# Autodesk Inventor assembly: Złożenie całości
(part 2 of 2)
- Wstaw:98 [Insert]: Prowadnica liniowa typu MGN12H 600mm:1 ↔ CNS 3932 M 3 x 5:80
- Wstaw:99 [Insert]: Prowadnica liniowa typu MGN12H 600mm:1 ↔ CNS 3932 M 3 x 5:81
- Wstaw:100 [Insert]: Prowadnica liniowa typu MGN12H 600mm:1 ↔ CNS 3932 M 3 x 5:82
- Wstaw:101 [Insert]: Prowadnica liniowa typu MGN12H 600mm:1 ↔ CNS 3932 M 3 x 5:83
- Wstaw:102 [Insert]: Prowadnica liniowa typu MGN12H 600mm:1 ↔ CNS 3932 M 3 x 5:84
- Zestawiający:70 [Mate]: Prowadnica liniowa typu MGN12H 600mm:2 ↔ Wózek MGN12H:1
- Zestawiający:71 [Mate]: Prowadnica liniowa typu MGN12H 600mm:2 ↔ Wózek MGN12H:1
- Zestawiający:72 [Mate]: Prowadnica liniowa typu MGN12H 600mm:1 ↔ Wózek MGN12H:2
- Zestawiający:73 [Mate]: Prowadnica liniowa typu MGN12H 600mm:1 ↔ Wózek MGN12H:2
- Równoległy:56 [Flush]: Wózek MGN12H:1 ↔ Wózek MGN12H:2
- Zestawiający:77 [Mate]: Profil dolny posuwu osi Y:1 ↔ Wspornik pionowy osi Y - lewa strona:1
- Równoległy:57 [Flush]: Profil dolny posuwu osi Y:1 ↔ Wspornik pionowy osi Y - lewa strona:1
- Równoległy:58 [Flush]: Profil dolny posuwu osi Y:1 ↔ Wspornik pionowy osi Y - lewa strona:1
- Zestawiający:78 [Mate]: Łożysko kulowe jednorzędowe 6200 2RS:1 ↔ Wspornik pionowy osi Y - lewa strona:1
- Równoległy:59 [Flush]: Łożysko kulowe jednorzędowe 6200 2RS:1 ↔ Wspornik pionowy osi Y - lewa strona:1
- Zestawiający:79 [Mate]: Profil dolny posuwu osi Y:1 ↔ Wspornik pionowy osi Y - prawa strona:1
- Równoległy:60 [Flush]: Profil dolny posuwu osi Y:1 ↔ Wspornik pionowy osi Y - prawa strona:1
- Równoległy:61 [Flush]: Profil dolny posuwu osi Y:1 ↔ Wspornik pionowy osi Y - prawa strona:1
- Równoległy:63 [Flush]: Profil aluminiowy alutec K&K 104080:1 ↔ Prowadnica liniowa typu MGN12H 600mm:2
- Równoległy:64 [Flush]: Profil aluminiowy alutec K&K 104080:1 ↔ Prowadnica liniowa typu MGN12H 600mm:1
- Zestawiający:80 [Mate]: Wózek MGN9C:1 ↔ Wspornik pionowy osi Y - lewa strona:1
- Zestawiający:81 [Mate]: Wózek MGN9C:2 ↔ Wspornik pionowy osi Y - lewa strona:1
- Zestawiający:82 [Mate]: Wózek MGN9C:3 ↔ Wspornik pionowy osi Y - prawa strona:1
- Zestawiający:83 [Mate]: Wózek MGN9C:4 ↔ Wspornik pionowy osi Y - prawa strona:1
- Zestawiający:84 [Mate]: Profil aluminiowy alutec K&K 104080:1 ↔ Wspornik pionowy osi Y - prawa strona:1
- Równoległy:65 [Flush] (70 mm): Profil aluminiowy alutec K&K 104080:1 ↔ Wspornik pionowy osi Y - prawa strona:1
- Równoległy:66 [Flush]: Profil aluminiowy alutec K&K 104080:1 ↔ Wspornik pionowy osi Y - prawa strona:1
- Zestawiający:94 [Mate] (70 mm): Wrzeciono Elektrowrzeciono CNC 0.8kw:1 ↔ Sklejka stołu:1
- Równoległy:67 [Flush]: Wspornik pionowy osi Y - prawa strona:1 ↔ Wspornik łożyska osi Y - prawa strona:1
- Zestawiający:97 [Mate]: Wspornik pionowy osi Y - prawa strona:1 ↔ Wspornik łożyska osi Y - prawa strona:1
- Równoległy:68 [Flush]: Wspornik pionowy osi Y - prawa strona:1 ↔ Wspornik łożyska osi Y - prawa strona:1
- Zestawiający:106 [Mate]: Wspornik pionowy osi Z:1 ↔ Obudowa nakrętki trapezowej fi 16:2
- Zestawiający:107 [Mate]: Wspornik pionowy osi Z:1 ↔ Obudowa nakrętki trapezowej fi 16:2
- Zestawiający:108 [Mate]: Wspornik pionowy osi Z:1 ↔ Obudowa nakrętki trapezowej fi 16:2
- Zestawiający:109 [Mate]: Nakrętka trapezowa kołnierzowa JFRM-2835TR16x4:2 ↔ Obudowa nakrętki trapezowej fi 16:2
- Zestawiający:110 [Mate]: Nakrętka trapezowa kołnierzowa JFRM-2835TR16x4:2 ↔ Obudowa nakrętki trapezowej fi 16:2
- Zestawiający:111 [Mate]: Nakrętka trapezowa kołnierzowa JFRM-2835TR16x4:2 ↔ Obudowa nakrętki trapezowej fi 16:2
- Zestawiający:112 [Mate]: Nakrętka trapezowa kołnierzowa JFRM-2835TR16x4:1 ↔ Obudowa nakrętki trapezowej fi 16:1
- Wstaw:111 [Insert]: Nakrętka trapezowa kołnierzowa JFRM-2835TR16x4:2 ↔ CNS 3932 M 5 x 10:9
- Wstaw:112 [Insert]: Nakrętka trapezowa kołnierzowa JFRM-2835TR16x4:2 ↔ CNS 3932 M 5 x 10:10
- Wstaw:113 [Insert]: Nakrętka trapezowa kołnierzowa JFRM-2835TR16x4:2 ↔ CNS 3932 M 5 x 10:11
- Wstaw:114 [Insert]: Nakrętka trapezowa kołnierzowa JFRM-2835TR16x4:2 ↔ CNS 3932 M 5 x 10:12
- Wstaw:115 [Insert]: Nakrętka trapezowa kołnierzowa JFRM-2835TR16x4:2 ↔ CNS 3932 M 5 x 10:13
- Wstaw:116 [Insert]: Nakrętka trapezowa kołnierzowa JFRM-2835TR16x4:2 ↔ CNS 3932 M 5 x 10:14
- Wstaw:117 [Insert]: Nakrętka trapezowa kołnierzowa JFRM-2835TR16x4:1 ↔ CNS 3932 M 5 x 10:15
- Wstaw:118 [Insert]: Nakrętka trapezowa kołnierzowa JFRM-2835TR16x4:1 ↔ CNS 3932 M 5 x 10:16
- Wstaw:119 [Insert]: Nakrętka trapezowa kołnierzowa JFRM-2835TR16x4:1 ↔ CNS 3932 M 5 x 10:17
- Wstaw:120 [Insert]: Nakrętka trapezowa kołnierzowa JFRM-2835TR16x4:1 ↔ CNS 3932 M 5 x 10:18
- Wstaw:121 [Insert]: Nakrętka trapezowa kołnierzowa JFRM-2835TR16x4:1 ↔ CNS 3932 M 5 x 10:19
- Wstaw:122 [Insert]: Nakrętka trapezowa kołnierzowa JFRM-2835TR16x4:1 ↔ CNS 3932 M 5 x 10:20
- Wstaw:123 [Insert]: Obudowa nakrętki trapezowej fi 16:2 ↔ CNS 3932 M 5 x 12:5
- Wstaw:124 [Insert]: Obudowa nakrętki trapezowej fi 16:2 ↔ CNS 3932 M 5 x 12:8
- Wstaw:125 [Insert]: Obudowa nakrętki trapezowej fi 16:2 ↔ CNS 3932 M 5 x 12:6
- Wstaw:126 [Insert]: Obudowa nakrętki trapezowej fi 16:2 ↔ CNS 3932 M 5 x 12:7
- Wstaw:127 [Insert]: Tuleja zaciskowo rozprężna RCK BK 80 8x15 Clampex:2 ↔ CNS 3932 M 4 x 6:7
- Wstaw:128 [Insert]: Tuleja zaciskowo rozprężna RCK BK 80 8x15 Clampex:2 ↔ CNS 3932 M 4 x 6:8
- Wstaw:129 [Insert]: Tuleja zaciskowo rozprężna RCK BK 80 8x15 Clampex:2 ↔ CNS 3932 M 4 x 6:9
- Wstaw:130 [Insert]: Tuleja zaciskowo rozprężna RCK BK 80 8x15 Clampex:2 ↔ CNS 3932 M 4 x 6:10
- Wstaw:131 [Insert]: Tuleja zaciskowo rozprężna RCK BK 80 8x15 Clampex:2 ↔ CNS 3932 M 4 x 6:11
- Wstaw:132 [Insert]: Tuleja zaciskowo rozprężna RCK BK 80 8x15 Clampex:2 ↔ CNS 3932 M 4 x 6:12
- Zestawiający:118 [Mate]: Silnik krokowy SM 60 100-4004AF - 4Nm:2 ↔ Koło zębate 21 T5 14 2F:2
- Zestawiający:119 [Mate] (1 mm): Silnik krokowy SM 60 100-4004AF - 4Nm:2 ↔ Koło zębate 21 T5 14 2F:2
- Zestawiający:120 [Mate] (18 mm): Wspornik pionowy osi Y - prawa strona:1 ↔ Silnik krokowy SM 60 100-4004AF - 4Nm:2
- Wstaw:133 [Insert]: Wspornik pionowy osi Y - lewa strona:1 ↔ CNS 3932 M 8 x 14:1
- Wstaw:134 [Insert]: Wspornik pionowy osi Y - lewa strona:1 ↔ CNS 3932 M 8 x 14:2
- Wstaw:135 [Insert]: Wspornik pionowy osi Y - prawa strona:1 ↔ CNS 3932 M 8 x 14:3
- Wstaw:136 [Insert]: Wspornik pionowy osi Y - prawa strona:1 ↔ CNS 3932 M 8 x 14:4
- Zestawiający:135 [Mate]: Profil dolny długi:2 ↔ Profil dolny krótki:2
- Wstaw:145 [Insert]: Wspornik pionowy osi Y - prawa strona:1 ↔ CNS 3932 M 4 x 6:21
- Wstaw:146 [Insert]: Wspornik pionowy osi Y - prawa strona:1 ↔ CNS 3932 M 4 x 6:22
- Wstaw:147 [Insert]: Wspornik pionowy osi Y - prawa strona:1 ↔ CNS 3932 M 4 x 6:23
- Wstaw:148 [Insert]: Wspornik pionowy osi Y - prawa strona:1 ↔ CNS 3932 M 4 x 6:24
- Wstaw:149 [Insert]: Wspornik pionowy osi Y - prawa strona:1 ↔ CNS 3932 M 4 x 6:25
- Wstaw:150 [Insert]: Wspornik pionowy osi Y - prawa strona:1 ↔ CNS 3932 M 4 x 6:26
- Wstaw:151 [Insert]: Wspornik pionowy osi Y - prawa strona:1 ↔ CNS 3932 M 4 x 6:27
- Wstaw:152 [Insert]: Wspornik pionowy osi Y - prawa strona:1 ↔ CNS 3932 M 4 x 6:28
- Zestawiający:139 [Mate]: Wspornik pionowy osi Y - prawa strona:1 ↔ CNS 3932 M 4 x 16:1
- Zestawiający:141 [Mate]: Wspornik pionowy osi Y - prawa strona:1 ↔ CNS 3932 M 4 x 16:2
- Zestawiający:143 [Mate]: Wspornik pionowy osi Y - prawa strona:1 ↔ CNS 3932 M 4 x 16:3
- Zestawiający:145 [Mate]: Wspornik pionowy osi Y - prawa strona:1 ↔ CNS 3932 M 4 x 16:4
- Wstaw:153 [Insert]: Silnik krokowy SM 60 100-4004AF - 4Nm:2 ↔ CNS 3932 M 5 x 12:10
- Wstaw:154 [Insert]: Silnik krokowy SM 60 100-4004AF - 4Nm:2 ↔ CNS 3932 M 5 x 12:11
- Wstaw:155 [Insert]: Silnik krokowy SM 60 100-4004AF - 4Nm:2 ↔ CNS 3932 M 5 x 12:12
- Wstaw:156 [Insert]: Silnik krokowy SM 60 100-4004AF - 4Nm:2 ↔ CNS 3932 M 5 x 12:13
- Zestawiający:146 [Mate]: CNS 3932 M 5 x 12:12 ↔ Uchwyt silnika krokowego osi X - płaski:1
- Zestawiający:147 [Mate]: CNS 3932 M 5 x 12:13 ↔ Uchwyt silnika krokowego osi X - płaski:1
- Zestawiający:148 [Mate]: Silnik krokowy SM 60 100-4004AF - 4Nm:2 ↔ Uchwyt silnika krokowego osi X - płaski:1
- Zestawiający:150 [Mate]: Wspornik pionowy osi Y - prawa strona:1 ↔ Uchwyt silnika krokowego osi X - płaski:1
- Zestawiający:151 [Mate]: Koło zębate 21 T5 28 2F:2 ↔ Tuleja zaciskowo rozprężna RCK BK 80 8x15 Clampex:2
- Zestawiający:152 [Mate]: Koło zębate 21 T5 28 2F:2 ↔ Tuleja zaciskowo rozprężna RCK BK 80 8x15 Clampex:2
- Zestawiający:153 [Mate]: Łożysko kulowe jednorzędowe 6200 2RS:1 ↔ Śruba trapezowa 16x4 - oś X:1
- Zestawiający:154 [Mate]: Łożysko kulowe jednorzędowe 6200 2RS:1 ↔ Śruba trapezowa 16x4 - oś X:1
- Zestawiający:155 [Mate]: Łożysko kulowe jednorzędowe 3200 2RS:1 ↔ Śruba trapezowa 16x4 - oś X:1
- Zestawiający:156 [Mate]: Łożysko kulowe jednorzędowe 3200 2RS:1 ↔ Śruba trapezowa 16x4 - oś X:1
- Zestawiający:157 [Mate]: Śruba trapezowa 16x4 - oś X:1 ↔ Tuleja zaciskowo rozprężna RCK BK 80 8x15 Clampex:2
- Równoległy:69 [Flush]: Koło zębate 21 T5 28 2F:2 ↔ Koło zębate 21 T5 14 2F:2
- Wstaw:157 [Insert]: Wspornik łożyska osi Y - prawa strona:1 ↔ CNS 3932 M 4 x 22:1
- Wstaw:158 [Insert]: Wspornik łożyska osi Y - prawa strona:1 ↔ CNS 3932 M 4 x 22:2
- Wstaw:159 [Insert]: Wspornik łożyska osi Y - prawa strona:1 ↔ CNS 3932 M 4 x 22:3
- Wstaw:160 [Insert]: Wspornik łożyska osi Y - prawa strona:1 ↔ CNS 3932 M 4 x 22:4
- Zestawiający:158 [Mate]: Koło zębate 21 T5 28 2F:2 ↔ Pas zębaty 10 T5-305:1
- Zestawiający:159 [Mate]: Koło zębate 21 T5 28 2F:2 ↔ Pas zębaty 10 T5-305:1
- Zestawiający:160 [Mate]: Koło zębate 21 T5 14 2F:2 ↔ Pas zębaty 10 T5-305:1
- Równoległy:70 [Flush] (2 mm): Profil dolny krótki:1 ↔ Łożysko w obudowie aluminiowej 10mm KP000:2
- Zestawiający:161 [Mate] (236.5 mm): Profil dolny długi:2 ↔ Łożysko w obudowie aluminiowej 10mm KP000:2
- Zestawiający:162 [Mate]: Śruba trapezowa 16x4:1 ↔ Obudowa nakrętki trapezowej fi 16:1
- Zestawiający:163 [Mate]: Nakrętka trapezowa kołnierzowa JFRM-2835TR16x4:1 ↔ Obudowa nakrętki trapezowej fi 16:1
- Zestawiający:164 [Mate]: Śruba trapezowa 16x4:1 ↔ Łożysko kulowe jednorzędowe 3200 2RS:2
- Zestawiający:165 [Mate]: Śruba trapezowa 16x4:1 ↔ Łożysko kulowe jednorzędowe 3200 2RS:2
- Zestawiający:169 [Mate]: DIN 6926 - zastąpiona przez DIN EN 1663/1666 M10:1 ↔ Łożysko kulowe jednorzędowe 3200 2RS:2
- Zestawiający:170 [Mate]: Sklejka stołu:1 ↔ Uchwyt łożyska wałka trapezowego osi Y:1
- Zestawiający:171 [Mate]: Śruba trapezowa 16x4:1 ↔ Uchwyt łożyska wałka trapezowego osi Y:1
- Zestawiający:172 [Mate]: Profil dolny krótki:2 ↔ Uchwyt łożyska wałka trapezowego osi Y:1
- Zestawiający:173 [Mate]: Koło zębate 21 T5 14 2F:1 ↔ Uchwyt silnika krokowego osi Y - płaski:1
- Zestawiający:174 [Mate]: Silnik krokowy SM 60 100-4004AF - 4Nm:1 ↔ Uchwyt silnika krokowego osi Y - płaski:1
- Równoległy:71 [Flush]: Silnik krokowy SM 60 100-4004AF - 4Nm:1 ↔ Uchwyt silnika krokowego osi Y - płaski:1
- Zestawiający:175 [Mate]: Sklejka stołu:1 ↔ Uchwyt silnika krokowego osi Y - płaski:1
- Zestawiający:176 [Mate]: Profil dolny krótki:2 ↔ Uchwyt silnika krokowego osi Y - płaski:1
- Równoległy:72 [Flush]: Koło zębate 21 T5 28 2F:1 ↔ Koło zębate 21 T5 14 2F:1
- Zestawiający:177 [Mate]: Tuleja zaciskowo rozprężna RCK BK 80 8x15 Clampex:1 ↔ Pas zębaty 10 T5-305:2
- Zestawiający:178 [Mate]: Koło zębate 21 T5 28 2F:1 ↔ Pas zębaty 10 T5-305:2
- Zestawiający:179 [Mate]: Koło zębate 21 T5 14 2F:1 ↔ Pas zębaty 10 T5-305:2
- Wstaw:165 [Insert]: Uchwyt silnika krokowego osi Y - płaski:1 ↔ CNS 3932 M 5 x 10:21
- Wstaw:166 [Insert]: Uchwyt silnika krokowego osi Y - płaski:1 ↔ CNS 3932 M 5 x 10:22
- Wstaw:167 [Insert]: Uchwyt silnika krokowego osi Y - płaski:1 ↔ CNS 3932 M 5 x 10:23
- Wstaw:168 [Insert]: Uchwyt silnika krokowego osi Y - płaski:1 ↔ CNS 3932 M 5 x 10:24
- Wstaw:169 [Insert]: Uchwyt łożyska wałka trapezowego osi Y:1 ↔ CNS 3932 M 4 x 6:29
- Wstaw:170 [Insert]: Uchwyt łożyska wałka trapezowego osi Y:1 ↔ CNS 3932 M 4 x 6:30
- Wstaw:171 [Insert]: Uchwyt łożyska wałka trapezowego osi Y:1 ↔ CNS 3932 M 4 x 6:31
- Wstaw:172 [Insert]: Uchwyt łożyska wałka trapezowego osi Y:1 ↔ CNS 3932 M 4 x 6:32
- Wstaw:173 [Insert]: Uchwyt łożyska wałka trapezowego osi Y:1 ↔ CNS 3932 M 4 x 6:33
- Wstaw:174 [Insert]: Uchwyt łożyska wałka trapezowego osi Y:1 ↔ CNS 3932 M 4 x 6:34
- Wstaw:175 [Insert]: Uchwyt łożyska wałka trapezowego osi Y:1 ↔ CNS 3932 M 4 x 6:35
- Wstaw:176 [Insert]: Uchwyt łożyska wałka trapezowego osi Y:1 ↔ CNS 3932 M 4 x 6:36
- Wstaw:177 [Insert]: Wspornik pionowy osi Y - lewa strona:1 ↔ CNS 3932 M 5 x 10:25
- Wstaw:178 [Insert]: Wspornik pionowy osi Y - lewa strona:1 ↔ CNS 3932 M 5 x 10:26
- Wstaw:179 [Insert]: Wspornik pionowy osi Y - prawa strona:1 ↔ CNS 3932 M 5 x 10:27
- Wstaw:180 [Insert]: Wspornik pionowy osi Y - prawa strona:1 ↔ CNS 3932 M 5 x 10:28
- Zestawiający:180 [Mate]: Wspornik pionowy osi Z:1 ↔ DIN 7991 M3x8:1
- Zestawiający:181 [Mate]: Wspornik pionowy osi Z:1 ↔ DIN 7991 M3x8:2
- Zestawiający:182 [Mate]: Wspornik pionowy osi Z:1 ↔ DIN 7991 M3x8:3
- Zestawiający:183 [Mate]: Wspornik pionowy osi Z:1 ↔ DIN 7991 M3x8:4
- Zestawiający:184 [Mate]: Wspornik pionowy osi Z:1 ↔ DIN 7991 M3x8:5
- Zestawiający:185 [Mate]: Wspornik pionowy osi Z:1 ↔ DIN 7991 M3x8:6
- Zestawiający:186 [Mate]: Wspornik pionowy osi Z:1 ↔ DIN 7991 M3x8:7
- Zestawiający:187 [Mate]: Wspornik pionowy osi Z:1 ↔ DIN 7991 M3x8:8
- Zestawiający:188 [Mate]: Wózek MGN12H:1 ↔ Wspornik pionowy osi Z:1
- Zestawiający:189 [Mate]: Wózek MGN12H:2 ↔ Wspornik pionowy osi Z:1
- Zestawiający:190 [Mate]: Wózek MGN12H:1 ↔ Wspornik pionowy osi Z:1
- Zestawiający:201 [Mate]: Pręt liniowy osi Z:1 ↔ Łożysko liniowe w obudowie SMAG10UU-L:2
- Zestawiający:202 [Mate]: Łożysko liniowe w obudowie SMAG10UU-L:1 ↔ Pręt liniowy osi Z:2
- Równoległy:75 [Flush]: Łożysko liniowe w obudowie SMAG10UU-L:1 ↔ Łożysko liniowe w obudowie SMAG10UU-L:2
- Równoległy:76 [Flush]: Łożysko liniowe w obudowie SMAG10UU-L:1 ↔ Łożysko liniowe w obudowie SMAG10UU-L:2
- Zestawiający:210 [Mate]: Nakrętka trapezowa kołnierzowa JFRM-2525TR10x3:1 ↔ Obudowa nakrętki trapezowej fi 10:1
- Zestawiający:211 [Mate]: Nakrętka trapezowa kołnierzowa JFRM-2525TR10x3:1 ↔ Obudowa nakrętki trapezowej fi 10:1
- Zestawiający:212 [Mate]: Nakrętka trapezowa kołnierzowa JFRM-2525TR10x3:1 ↔ Obudowa nakrętki trapezowej fi 10:1
- Wstaw:181 [Insert]: Nakrętka trapezowa kołnierzowa JFRM-2525TR10x3:1 ↔ CNS 3932 M 5 x 20:1
- Wstaw:182 [Insert]: Nakrętka trapezowa kołnierzowa JFRM-2525TR10x3:1 ↔ CNS 3932 M 5 x 20:2
- Wstaw:183 [Insert]: Nakrętka trapezowa kołnierzowa JFRM-2525TR10x3:1 ↔ CNS 3932 M 5 x 20:3
- Wstaw:184 [Insert]: Nakrętka trapezowa kołnierzowa JFRM-2525TR10x3:1 ↔ CNS 3932 M 5 x 20:4
- Wstaw:185 [Insert]: Nakrętka trapezowa kołnierzowa JFRM-2525TR10x3:1 ↔ CNS 3932 M 5 x 20:5
- Wstaw:186 [Insert]: Nakrętka trapezowa kołnierzowa JFRM-2525TR10x3:1 ↔ CNS 3932 M 5 x 20:6
- Zestawiający:213 [Mate]: Nakrętka trapezowa kołnierzowa JFRM-2525TR10x3:1 ↔ Śruba trapezowa 10x2 - oś Z:1
- Zestawiający:216 [Mate]: Śruba trapezowa 10x2 - oś Z:1 ↔ Łożysko kulowe jednorzędowe 6200 2RS:2
- Równoległy:81 [Flush]: Śruba trapezowa 10x2 - oś Z:1 ↔ Łożysko kulowe jednorzędowe 6200 2RS:2
- Równoległy:82 [Flush]: Łożysko liniowe w obudowie SMAG10UU-L:1 ↔ Obudowa nakrętki trapezowej fi 10:1
- Zestawiający:222 [Mate] (5 mm): Obudowa nakrętki trapezowej fi 16:2 ↔ Silnik krokowy SM 5776-2804MA - 1.89Nm:1
- Zestawiający:223 [Mate]: Silnik krokowy SM 5776-2804MA - 1.89Nm:1 ↔ Koło zębate 21 T5 14 2F:3
- Zestawiający:228 [Mate]: Podstawa górna osi Z:1 ↔ Łożysko kulowe jednorzędowe 3200 2RS:3
- Równoległy:84 [Flush] (10 mm): Podstawa górna osi Z:1 ↔ Łożysko kulowe jednorzędowe 3200 2RS:3
- Zestawiający:229 [Mate]: Śruba trapezowa 10x2 - oś Z:1 ↔ Łożysko kulowe jednorzędowe 3200 2RS:3
- Zestawiający:230 [Mate]: Wspornik pionowy osi Z:1 ↔ Podstawa górna osi Z:1
- Równoległy:85 [Flush]: Wspornik pionowy osi Z:1 ↔ Podstawa górna osi Z:1
- Wstaw:187 [Insert]: Podstawa górna osi Z:1 ↔ CNS 3932 M 4 x 16:5
- Wstaw:188 [Insert]: Podstawa górna osi Z:1 ↔ CNS 3932 M 4 x 16:6
- Wstaw:189 [Insert]: Wspornik pionowy osi Z:1 ↔ CNS 3932 M 5 x 25:1
- Wstaw:190 [Insert]: Wspornik pionowy osi Z:1 ↔ CNS 3932 M 5 x 25:2
- Wstaw:191 [Insert]: Wspornik pionowy osi Z:1 ↔ CNS 3932 M 5 x 25:3
- Wstaw:192 [Insert]: Wspornik pionowy osi Z:1 ↔ CNS 3932 M 5 x 25:4
- Zestawiający:231 [Mate]: Wspornik pionowy osi Z:1 ↔ Podstawa dolna osi Z:1
- Równoległy:86 [Flush]: Wspornik pionowy osi Z:1 ↔ Podstawa dolna osi Z:1
- Równoległy:87 [Flush]: Wspornik pionowy osi Z:1 ↔ Podstawa dolna osi Z:1
- Równoległy:88 [Flush]: Łożysko kulowe jednorzędowe 6200 2RS:2 ↔ Podstawa dolna osi Z:1
- Równoległy:89 [Flush]: Wspornik pionowy osi Z:1 ↔ Podstawa górna osi Z:1
- Równoległy:90 [Flush]: Pręt liniowy osi Z:2 ↔ Podstawa dolna osi Z:1
- Równoległy:91 [Flush]: Pręt liniowy osi Z:1 ↔ Podstawa dolna osi Z:1
- Zestawiający:232 [Mate]: Pręt liniowy osi Z:1 ↔ Podstawa dolna osi Z:1
- Zestawiający:233 [Mate]: Pręt liniowy osi Z:2 ↔ Podstawa dolna osi Z:1
- Wstaw:193 [Insert]: Podstawa dolna osi Z:1 ↔ CNS 3932 M 4 x 16:7
- Wstaw:194 [Insert]: Podstawa dolna osi Z:1 ↔ CNS 3932 M 4 x 16:8
- Zestawiający:234 [Mate]: Śruba trapezowa 10x2 - oś Z:1 ↔ Nakrętka trapezowa 10x17:2
- Zestawiający:236 [Mate]: Śruba trapezowa 10x2 - oś Z:1 ↔ Nakrętka trapezowa 10x17:1
- Zestawiający:237 [Mate]: Śruba trapezowa 10x2 - oś Z:1 ↔ DIN 433-1 A 10,5:1
- Zestawiający:238 [Mate]: Łożysko kulowe jednorzędowe 3200 2RS:3 ↔ DIN 433-1 A 10,5:1
- Zestawiający:239 [Mate]: Nakrętka trapezowa 10x17:1 ↔ DIN 433-1 A 10,5:1
- Zestawiający:240 [Mate]: Śruba trapezowa 10x2 - oś Z:1 ↔ DIN 433-1 A 10,5:2
- Zestawiający:241 [Mate]: Łożysko kulowe jednorzędowe 3200 2RS:3 ↔ DIN 433-1 A 10,5:2
- Zestawiający:242 [Mate]: Nakrętka trapezowa 10x17:2 ↔ DIN 433-1 A 10,5:2
- Równoległy:92 [Flush]: Łożysko liniowe w obudowie SMAG10UU-L:1 ↔ Obudowa nakrętki trapezowej fi 10:1
- Zestawiający:243 [Mate]: Wspornik pionowy osi Z:1 ↔ Uchwyt górnego łożyska osi Z:1
- Zestawiający:244 [Mate]: Podstawa górna osi Z:1 ↔ Uchwyt górnego łożyska osi Z:1
- Zestawiający:245 [Mate]: Łożysko kulowe jednorzędowe 3200 2RS:3 ↔ Uchwyt górnego łożyska osi Z:1
- Wstaw:195 [Insert]: Uchwyt górnego łożyska osi Z:1 ↔ CNS 3932 M 5 x 22:1
- Zestawiający:246 [Mate]: Podstawa górna osi Z:1 ↔ CNS 3932 M 5 x 22:15
- Zestawiający:247 [Mate]: Uchwyt górnego łożyska osi Z:1 ↔ CNS 3932 M 5 x 22:15
- Zestawiający:248 [Mate]: Podstawa górna osi Z:1 ↔ CNS 3932 M 5 x 22:3
- Zestawiający:249 [Mate]: Uchwyt górnego łożyska osi Z:1 ↔ CNS 3932 M 5 x 22:3
- Równoległy:93 [Flush] (0.5 mm): Silnik krokowy SM 5776-2804MA - 1.89Nm:1 ↔ Koło zębate 21 T5 14 2F:3
- Zestawiający:250 [Mate]: Śruba trapezowa 10x2 - oś Z:1 ↔ Tuleja zaciskowo rozprężna RCK BK 80 10x16 Clampex:1
- Zestawiający:251 [Mate]: Tuleja zaciskowo rozprężna RCK BK 80 10x16 Clampex:1 ↔ Koło zębate 21 T5 28 2F - toczenie pod tuleję zaciskowo rozprężną fi 10:1
- Zestawiający:252 [Mate]: Tuleja zaciskowo rozprężna RCK BK 80 10x16 Clampex:1 ↔ Koło zębate 21 T5 28 2F - toczenie pod tuleję zaciskowo rozprężną fi 10:1
- Zestawiający:253 [Mate]: Tuleja zaciskowo rozprężna RCK BK 80 10x16 Clampex:1 ↔ CNS 3932 M 4 x 6:37
- Zestawiający:254 [Mate]: Tuleja zaciskowo rozprężna RCK BK 80 10x16 Clampex:1 ↔ CNS 3932 M 4 x 6:37
- Zestawiający:255 [Mate]: Tuleja zaciskowo rozprężna RCK BK 80 10x16 Clampex:1 ↔ CNS 3932 M 4 x 6:38
- Zestawiający:256 [Mate]: Tuleja zaciskowo rozprężna RCK BK 80 10x16 Clampex:1 ↔ CNS 3932 M 4 x 6:38
- Zestawiający:257 [Mate]: Tuleja zaciskowo rozprężna RCK BK 80 10x16 Clampex:1 ↔ CNS 3932 M 4 x 6:39
- Zestawiający:258 [Mate]: Tuleja zaciskowo rozprężna RCK BK 80 10x16 Clampex:1 ↔ CNS 3932 M 4 x 6:39
- Zestawiający:259 [Mate]: Tuleja zaciskowo rozprężna RCK BK 80 10x16 Clampex:1 ↔ CNS 3932 M 4 x 6:40
- Zestawiający:260 [Mate]: Tuleja zaciskowo rozprężna RCK BK 80 10x16 Clampex:1 ↔ CNS 3932 M 4 x 6:40
- Zestawiający:261 [Mate]: Tuleja zaciskowo rozprężna RCK BK 80 10x16 Clampex:1 ↔ CNS 3932 M 4 x 6:41
- Zestawiający:262 [Mate]: Tuleja zaciskowo rozprężna RCK BK 80 10x16 Clampex:1 ↔ CNS 3932 M 4 x 6:41
- Zestawiający:263 [Mate]: Tuleja zaciskowo rozprężna RCK BK 80 10x16 Clampex:1 ↔ CNS 3932 M 4 x 6:42
- Zestawiający:264 [Mate]: Tuleja zaciskowo rozprężna RCK BK 80 10x16 Clampex:1 ↔ CNS 3932 M 4 x 6:42
- Równoległy:94 [Flush]: Koło zębate 21 T5 14 2F:3 ↔ Koło zębate 21 T5 28 2F - toczenie pod tuleję zaciskowo rozprężną fi 10:1
- Równoległy:95 [Flush]: Silnik krokowy SM 5776-2804MA - 1.89Nm:1 ↔ Podstawa górna osi Z:1
- Zestawiający:265 [Mate] (15 mm): Wspornik pionowy osi Z:1 ↔ Silnik krokowy SM 5776-2804MA - 1.89Nm:1
- Zestawiający:266 [Mate]: Podstawa górna osi Z:1 ↔ Uchwyt silnika krokowego osi Z:1
- Równoległy:96 [Flush]: Podstawa górna osi Z:1 ↔ Uchwyt silnika krokowego osi Z:1
- Równoległy:97 [Flush]: Podstawa górna osi Z:1 ↔ Uchwyt silnika krokowego osi Z:1
- Zestawiający:267 [Mate]: Koło zębate 21 T5 28 2F - toczenie pod tuleję zaciskowo rozprężną fi 10:1 ↔ Pas zębaty 10 T5-275:1
- Zestawiający:268 [Mate]: Koło zębate 21 T5 14 2F:3 ↔ Pas zębaty 10 T5-275:1
- Zestawiający:269 [Mate]: Koło zębate 21 T5 14 2F:3 ↔ Pas zębaty 10 T5-275:1
- Zestawiający:270 [Mate]: Silnik krokowy SM 5776-2804MA - 1.89Nm:1 ↔ CNS 3932 M 5 x 22:7
- Zestawiający:271 [Mate]: CNS 3932 M 5 x 22:7 ↔ DIN 433-1 A 6,4:1
- Zestawiający:272 [Mate]: CNS 3932 M 5 x 22:7 ↔ DIN 433-1 A 6,4:1
- Zestawiający:273 [Mate]: Uchwyt silnika krokowego osi Z:1 ↔ DIN 433-1 A 6,4:1
- Zestawiający:274 [Mate]: CNS 3932 M 5 x 22:7 ↔ DIN 433-1 A 6,4:2
- Zestawiający:275 [Mate]: Silnik krokowy SM 5776-2804MA - 1.89Nm:1 ↔ DIN 433-1 A 6,4:2
- Zestawiający:276 [Mate]: CNS 3932 M 5 x 22:7 ↔ JIS B 1181 Styl 1 - Metryczny A M5:1
- Zestawiający:277 [Mate]: DIN 433-1 A 6,4:2 ↔ JIS B 1181 Styl 1 - Metryczny A M5:1
- Zestawiający:278 [Mate]: Silnik krokowy SM 5776-2804MA - 1.89Nm:1 ↔ CNS 3932 M 5 x 22:4
- Zestawiający:279 [Mate]: Silnik krokowy SM 5776-2804MA - 1.89Nm:1 ↔ CNS 3932 M 5 x 22:5
- Zestawiający:280 [Mate]: Silnik krokowy SM 5776-2804MA - 1.89Nm:1 ↔ CNS 3932 M 5 x 22:6
- Zestawiający:281 [Mate]: CNS 3932 M 5 x 22:6 ↔ DIN 433-1 A 6,4:3
- Zestawiający:282 [Mate]: CNS 3932 M 5 x 22:4 ↔ DIN 433-1 A 6,4:6
- Zestawiający:283 [Mate]: CNS 3932 M 5 x 22:5 ↔ DIN 433-1 A 6,4:7
- Zestawiający:284 [Mate]: CNS 3932 M 5 x 22:6 ↔ DIN 433-1 A 6,4:3
- Zestawiający:285 [Mate]: CNS 3932 M 5 x 22:4 ↔ DIN 433-1 A 6,4:6
- Zestawiający:286 [Mate]: CNS 3932 M 5 x 22:5 ↔ DIN 433-1 A 6,4:7
- Zestawiający:287 [Mate]: Uchwyt silnika krokowego osi Z:1 ↔ DIN 433-1 A 6,4:7
- Zestawiający:288 [Mate]: Uchwyt silnika krokowego osi Z:1 ↔ DIN 433-1 A 6,4:3
- Zestawiający:289 [Mate]: Uchwyt silnika krokowego osi Z:1 ↔ DIN 433-1 A 6,4:6
- Zestawiający:290 [Mate]: CNS 3932 M 5 x 22:4 ↔ DIN 433-1 A 6,4:4
- Zestawiający:291 [Mate]: Silnik krokowy SM 5776-2804MA - 1.89Nm:1 ↔ DIN 433-1 A 6,4:4
- Zestawiający:292 [Mate]: CNS 3932 M 5 x 22:6 ↔ DIN 433-1 A 6,4:5
- Zestawiający:293 [Mate]: Silnik krokowy SM 5776-2804MA - 1.89Nm:1 ↔ DIN 433-1 A 6,4:5
- Zestawiający:294 [Mate]: CNS 3932 M 5 x 22:5 ↔ DIN 433-1 A 6,4:8
- Zestawiający:295 [Mate]: Silnik krokowy SM 5776-2804MA - 1.89Nm:1 ↔ DIN 433-1 A 6,4:8
- Zestawiający:296 [Mate]: CNS 3932 M 5 x 22:5 ↔ JIS B 1181 Styl 1 - Metryczny A M5:2
- Zestawiający:297 [Mate]: DIN 433-1 A 6,4:8 ↔ JIS B 1181 Styl 1 - Metryczny A M5:2
- Zestawiający:298 [Mate]: CNS 3932 M 5 x 22:4 ↔ JIS B 1181 Styl 1 - Metryczny A M5:3
- Zestawiający:299 [Mate]: DIN 433-1 A 6,4:4 ↔ JIS B 1181 Styl 1 - Metryczny A M5:3
- Zestawiający:300 [Mate]: CNS 3932 M 5 x 22:6 ↔ JIS B 1181 Styl 1 - Metryczny A M5:4
- Zestawiający:301 [Mate]: DIN 433-1 A 6,4:5 ↔ JIS B 1181 Styl 1 - Metryczny A M5:4
- Wstaw:196 [Insert]: Uchwyt silnika krokowego osi Z:1 ↔ CNS 3932 M 5 x 16:1
- Wstaw:197 [Insert]: Uchwyt silnika krokowego osi Z:1 ↔ CNS 3932 M 5 x 16:2
- Wstaw:198 [Insert]: Uchwyt silnika krokowego osi Z:1 ↔ CNS 3932 M 5 x 16:3
- Wstaw:199 [Insert]: Uchwyt silnika krokowego osi Z:1 ↔ CNS 3932 M 5 x 16:4
